# Autodesk Inventor assembly: XLN25P_M
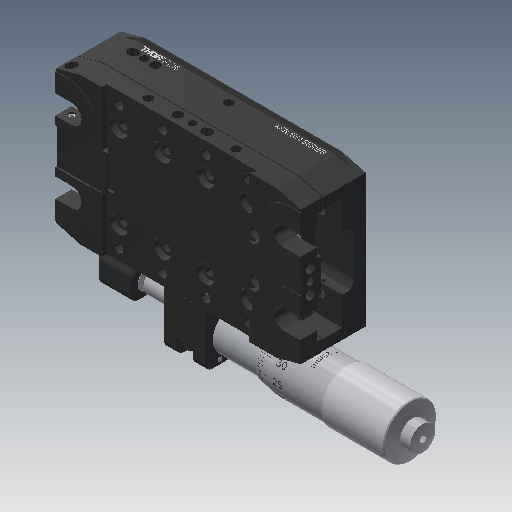
[picture p0: Inventor's stored thumbnail of the model, 512x512]
Saved by Autodesk Inventor 2019 (Build 230136000, 136)
## iProperties
Created: 2020-09-21
Part Number: XLN25P_M
Document SubType Name: Assembly
Designer: voigt
Author: voigt
## Documents named in this file (5)
- C:\Users\nvladi\Documents\Inventor\mesoSPIM_design_benchtop_V2\library\Thorlabs\stages\XLN25P_M.iam
- C:\Users\nvladi\Documents\Inventor\mesoSPIM_design_benchtop_V2\library\Thorlabs\stages\XLN25P_M_base.ipt
- C:\Users\nvladi\Documents\Inventor\mesoSPIM_design_benchtop_V2\library\Thorlabs\stages\XRN-B1_M-Micrometer-Micrometer-Counterplate.ipt
- C:\Users\nvladi\Documents\Inventor\mesoSPIM_design_benchtop_V2\library\Thorlabs\stages\XRN25P_M_Adjuster_Clamp.ipt
- C:\Users\nvladi\Documents\Inventor\mesoSPIM_design_benchtop_V2\library\Thorlabs\stages\XRN25P_M_Adjuster.ipt
## Components (4 placed, 4 different names)
1. XLN25P_M_base:1 — Mate:1, Mate:2, Angle:1, Mate:3, Mate:4, Angle:2
2. XRN-B1_M-Micrometer-Micrometer-Counterplate:1 — Mate:1, Mate:2, Angle:1
3. XRN25P_M_Adjuster_Clamp:1 — Mate:3, Mate:4, Angle:2, Mate:5, Mate:6
4. XRN25P_M_Adjuster:1 — Mate:5, Mate:6
## Relationships (8: Mate 6, Angle 2)
- Mate:1: XLN25P_M_base:1 ↔ XRN-B1_M-Micrometer-Micrometer-Counterplate:1
- Mate:2: XLN25P_M_base:1 ↔ XRN-B1_M-Micrometer-Micrometer-Counterplate:1
- Angle:1 (0 deg): XLN25P_M_base:1 ↔ XRN-B1_M-Micrometer-Micrometer-Counterplate:1
- Mate:3: XLN25P_M_base:1 ↔ XRN25P_M_Adjuster_Clamp:1
- Mate:4: XLN25P_M_base:1 ↔ XRN25P_M_Adjuster_Clamp:1
- Angle:2 (0 deg): XLN25P_M_base:1 ↔ XRN25P_M_Adjuster_Clamp:1
- Mate:5: XRN25P_M_Adjuster_Clamp:1 ↔ XRN25P_M_Adjuster:1
- Mate:6: XRN25P_M_Adjuster_Clamp:1 ↔ XRN25P_M_Adjuster:1
